# Autodesk Inventor assembly: SHANK2
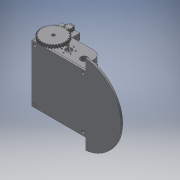
[picture p0: Inventor's stored thumbnail of the model, 180x180]
Saved by Autodesk Inventor 2019 (Build 230136000, 136)
## iProperties
Created: 2017-05-03
Part Number: SHANK2
Document SubType Name: Assembly
Designer: ANDRES
Author: ANDRES
## Documents named in this file (10)
- C:\Users\Andres\Documents\GitHub\Shank2.0\Variados\Diseño Mecanico\SHANK2.iam
- C:\Users\Andres\Documents\GitHub\Shank2.0\Variados\Diseño Mecanico\PCB_Final.ipt
- C:\Users\Andres\Documents\GitHub\Shank2.0\Variados\Diseño Mecanico\Base_Motor_acrilico_15.ipt
- C:\Users\Andres\Documents\GitHub\Shank2.0\Variados\Diseño Mecanico\Motor_Final.ipt
- C:\Users\Andres\Documents\GitHub\Shank2.0\Variados\Diseño Mecanico\Tornillo.ipt
- C:\Users\Andres\Documents\GitHub\Shank2.0\Variados\Diseño Mecanico\Spoiler.ipt
- C:\Users\Andres\Documents\GitHub\Shank2.0\Variados\Diseño Mecanico\Engranajes\Engranajes GRANDE final 2017.ipt
- C:\Users\Andres\Documents\GitHub\Shank2.0\Variados\Diseño Mecanico\encoder_engranaje.ipt
- C:\Users\Andres\Documents\GitHub\Shank2.0\Variados\Diseño Mecanico\Base_encoder.ipt
- C:\Users\Andres\Documents\GitHub\Shank2.0\Variados\Diseño Mecanico\Part2.ipt
## Components (11 placed, 9 different names)
1. PCB_Final:1 — Mate:1, Mate:2, Mate:3, Flush:1, Mate:5, Flush:2, Mate:8
2. Base_Motor_acrilico_15:1 — Mate:2, Flush:2, Mate:8, Flush:3, Cylindrical:3
3. Base_Motor_acrilico_15:2 — Mate:3, Flush:1, Mate:5, Cylindrical:1, Mate:7, Cylindrical:4
4. Motor_Final:1 — Cylindrical:1, Mate:6, Cylindrical:2, Mate:7
5. Motor_Final:2 — Mate:6, Cylindrical:2
6. Tornillo:1 — Flush:3, Cylindrical:3
7. Spoiler:1 — Flush:5, Flush:6
8. Engranajes GRANDE final 2017:1 — Cylindrical:4, Flush:4
9. encoder_engranaje:1 — Flush:4
10. Base_encoder:1 — Flush:5, Mate:9
11. Part2:1 — Flush:6, Mate:9
## Relationships (18: Mate 8, Flush 6, CylindricalJoint 4)
- Mate:1: PCB_Final:1
- Mate:2: PCB_Final:1 ↔ Base_Motor_acrilico_15:1
- Mate:3: PCB_Final:1 ↔ Base_Motor_acrilico_15:2
- Flush:1: PCB_Final:1 ↔ Base_Motor_acrilico_15:2
- Mate:5: PCB_Final:1 ↔ Base_Motor_acrilico_15:2
- Cylindrical:1: Base_Motor_acrilico_15:2 ↔ Motor_Final:1
- Mate:6: Motor_Final:1 ↔ Motor_Final:2
- Cylindrical:2: Motor_Final:1 ↔ Motor_Final:2
- Mate:7: Base_Motor_acrilico_15:2 ↔ Motor_Final:1
- Flush:2: PCB_Final:1 ↔ Base_Motor_acrilico_15:1
- Mate:8: PCB_Final:1 ↔ Base_Motor_acrilico_15:1
- Flush:3: Base_Motor_acrilico_15:1 ↔ Tornillo:1
- Cylindrical:3: Base_Motor_acrilico_15:1 ↔ Tornillo:1
- Cylindrical:4: Base_Motor_acrilico_15:2 ↔ Engranajes GRANDE final 2017:1
- Flush:4: Engranajes GRANDE final 2017:1 ↔ encoder_engranaje:1
- Flush:5: Spoiler:1 ↔ Base_encoder:1
- Flush:6: Spoiler:1 ↔ Part2:1
- Mate:9 (2 mm): Base_encoder:1 ↔ Part2:1
